# Autodesk Inventor assembly: Assignment 8 Arbor Press Assemblies
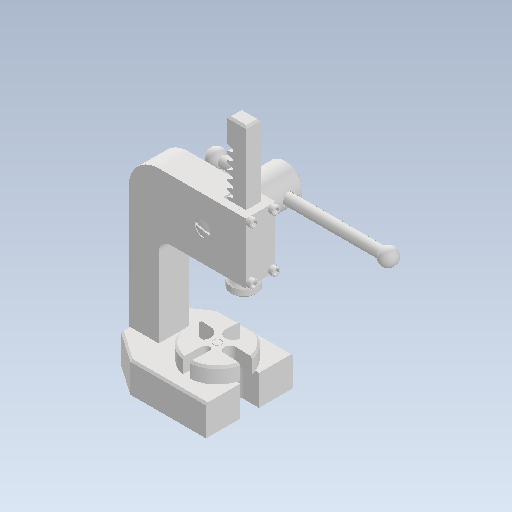
[picture p0: Inventor's stored thumbnail of the model, 512x512]
Saved by Autodesk Inventor 2020 (Build 240168000, 168)
## iProperties
Created: 2021-04-22
Part Number: Assignment 8 Arbor Press Assemblies
Document SubType Name: Assembly
Designer: austi
Author: austi
## Documents named in this file (15)
- D:\3D Modeling\Ch7(5)\Assignment 8 Arbor Press Assemblies.iam
- D:\3D Modeling\Ch7(5)\Ch7(5) Part 1 Base.ipt
- D:\3D Modeling\Ch7(5)\Imported Screw 191251A194_BLACK-OXIDE ALLOY STEEL SOCKET HEAD CAP SCREW.ipt
- D:\3D Modeling\Ch7(5)\Ch7(5) Part 2 Table Pen.ipt
- D:\3D Modeling\Ch7(5)\Ch7(5) Part 3 Table.ipt
- D:\3D Modeling\Ch7(5)\Ch7(5) Part 4 Ball End.ipt
- D:\3D Modeling\Ch7(5)\Ch7(5) Part 5 Sleeve.ipt
- D:\3D Modeling\Ch7(5)\Ch7(5) Part 6 Handle.ipt
- D:\3D Modeling\Ch7(5)\Ch7(5) Part 7 Gear.ipt
- D:\3D Modeling\Ch7(5)\Ch7(5) Part 8 Rack Pad.ipt
- D:\3D Modeling\Ch7(5)\Ch7(5) Part 9 Cover Plate.ipt
- D:\3D Modeling\Ch7(5)\Ch7(5) Part 11 Rack.ipt
- D:\3D Modeling\Ch7(5)\Ch7(5) Part 12 Screw.ipt
- D:\3D Modeling\Ch7(5)\Ch7(5) Part 13 Column.ipt
- D:\3D Modeling\Ch7(5)\Imported Screw 291251A624_BLACK-OXIDE ALLOY STEEL SOCKET HEAD CAP SCREW.ipt
## Components (18 placed, 14 different names)
1. Ch7(5) Part 1 Base:1 — Mate:4, Mate:5, Mate:6, Mate:7, Flush:3
2. Imported Screw 191251A194_BLACK-OXIDE ALLOY STEEL SOCKET HEAD CAP SCREW:1 — Insert:5
3. Imported Screw 191251A194_BLACK-OXIDE ALLOY STEEL SOCKET HEAD CAP SCREW:2 — Insert:6
4. Imported Screw 191251A194_BLACK-OXIDE ALLOY STEEL SOCKET HEAD CAP SCREW:3 — Insert:7
5. Imported Screw 191251A194_BLACK-OXIDE ALLOY STEEL SOCKET HEAD CAP SCREW:4 — Insert:4
6. Ch7(5) Part 2 Table Pen:1 — Insert:3
7. Ch7(5) Part 3 Table:1 — Mate:4, Mate:5, Insert:3
8. Ch7(5) Part 4 Ball End:1 — Insert:2
9. Ch7(5) Part 5 Sleeve:1 — Angle:1, Angle:2, Mate:15, Mate:16
10. Ch7(5) Part 6 Handle:1 — Insert:1, Insert:2, Mate:16
11. Ch7(5) Part 7 Gear:1 — Angle:2, Mate:15, Insert:8, Insert:9, Flush:6
12. Ch7(5) Part 8 Rack Pad:1 — Mate:18, Mate:19
13. Ch7(5) Part 9 Cover Plate:1 — Mate:10, Flush:5, Mate:11, Insert:4, Insert:5, Insert:6, Insert:7, Flush:7
14. Ch7(5) Part 11 Rack:1 — Mate:17, Mate:18, Mate:19, Flush:7
15. Ch7(5) Part 12 Screw:1 — Insert:8
16. Ch7(5) Part 13 Column:1 — Mate:6, Mate:7, Flush:3, Mate:10, Flush:5, Mate:11, Angle:1, Insert:9, Flush:6, Mate:17, Angle:3, Insert:10
17. Ch7(5) Part 4 Ball End:2 — Insert:1
18. Imported Screw 291251A624_BLACK-OXIDE ALLOY STEEL SOCKET HEAD CAP SCREW:1 — Angle:3, Insert:10
## Relationships (28: Mate 11, Insert 10, Flush 4, Angle 3)
- Insert:1: Ch7(5) Part 6 Handle:1 ↔ Ch7(5) Part 4 Ball End:2
- Insert:2: Ch7(5) Part 4 Ball End:1 ↔ Ch7(5) Part 6 Handle:1
- Mate:4: Ch7(5) Part 1 Base:1 ↔ Ch7(5) Part 3 Table:1
- Mate:5: Ch7(5) Part 1 Base:1 ↔ Ch7(5) Part 3 Table:1
- Insert:3: Ch7(5) Part 2 Table Pen:1 ↔ Ch7(5) Part 3 Table:1
- Mate:6: Ch7(5) Part 1 Base:1 ↔ Ch7(5) Part 13 Column:1
- Mate:7: Ch7(5) Part 1 Base:1 ↔ Ch7(5) Part 13 Column:1
- Flush:3: Ch7(5) Part 1 Base:1 ↔ Ch7(5) Part 13 Column:1
- Mate:10: Ch7(5) Part 9 Cover Plate:1 ↔ Ch7(5) Part 13 Column:1
- Flush:5: Ch7(5) Part 9 Cover Plate:1 ↔ Ch7(5) Part 13 Column:1
- Mate:11: Ch7(5) Part 9 Cover Plate:1 ↔ Ch7(5) Part 13 Column:1
- Insert:4: Imported Screw 191251A194_BLACK-OXIDE ALLOY STEEL SOCKET HEAD CAP SCREW:4 ↔ Ch7(5) Part 9 Cover Plate:1
- Insert:5: Imported Screw 191251A194_BLACK-OXIDE ALLOY STEEL SOCKET HEAD CAP SCREW:1 ↔ Ch7(5) Part 9 Cover Plate:1
- Insert:6: Imported Screw 191251A194_BLACK-OXIDE ALLOY STEEL SOCKET HEAD CAP SCREW:2 ↔ Ch7(5) Part 9 Cover Plate:1
- Insert:7: Imported Screw 191251A194_BLACK-OXIDE ALLOY STEEL SOCKET HEAD CAP SCREW:3 ↔ Ch7(5) Part 9 Cover Plate:1
- Angle:1 (0 deg): Ch7(5) Part 5 Sleeve:1 ↔ Ch7(5) Part 13 Column:1
- Angle:2 (0 deg): Ch7(5) Part 5 Sleeve:1 ↔ Ch7(5) Part 7 Gear:1
- Mate:15: Ch7(5) Part 5 Sleeve:1 ↔ Ch7(5) Part 7 Gear:1
- Insert:8: Ch7(5) Part 7 Gear:1 ↔ Ch7(5) Part 12 Screw:1
- Insert:9: Ch7(5) Part 7 Gear:1 ↔ Ch7(5) Part 13 Column:1
- Flush:6: Ch7(5) Part 7 Gear:1 ↔ Ch7(5) Part 13 Column:1
- Mate:16: Ch7(5) Part 5 Sleeve:1 ↔ Ch7(5) Part 6 Handle:1
- Mate:17: Ch7(5) Part 11 Rack:1 ↔ Ch7(5) Part 13 Column:1
- Mate:18: Ch7(5) Part 8 Rack Pad:1 ↔ Ch7(5) Part 11 Rack:1
- Mate:19: Ch7(5) Part 8 Rack Pad:1 ↔ Ch7(5) Part 11 Rack:1
- Flush:7: Ch7(5) Part 9 Cover Plate:1 ↔ Ch7(5) Part 11 Rack:1
- Angle:3 (0 deg): Ch7(5) Part 13 Column:1 ↔ Imported Screw 291251A624_BLACK-OXIDE ALLOY STEEL SOCKET HEAD CAP SCREW:1
- Insert:10: Ch7(5) Part 13 Column:1 ↔ Imported Screw 291251A624_BLACK-OXIDE ALLOY STEEL SOCKET HEAD CAP SCREW:1
